# Autodesk Inventor assembly: painel
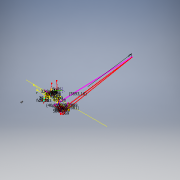
[picture p0: Inventor's stored thumbnail of the model, 180x180]
Saved by Autodesk Inventor 2019 (Build 230136000, 136)
## iProperties
Created: 2020-05-29
Part Number: painel
Document SubType Name: Assembly
Designer: luiza
_SolveAssemblyDoc: Frame Generator Solve Assembly
_Version: 15.0.0
Author: luiza
## Documents named in this file (8)
- G:\Meu Drive\Projetos\Projeto 2020 2021\Eletrônica 2020-2021\Projeção mecânica\Painel\old_painel.iam
- G:\Meu Drive\Projetos\Projeto 2020 2021\Eletrônica 2020-2021\Projeção mecânica\Painel\LCD12864_st7920.iam
- G:\Meu Drive\Projetos\Projeto 2020 2021\Eletrônica 2020-2021\Projeção mecânica\Painel\Tampa Painel.ipt
- G:\Meu Drive\Projetos\Projeto 2020 2021\Eletrônica 2020-2021\Projeção mecânica\Painel\Caixa Painel.ipt
- G:\Meu Drive\Projetos\Projeto 2020 2021\Eletrônica 2020-2021\Projeção mecânica\Painel\Espaçadores.ipt
- G:\Meu Drive\Projetos\Projeto 2020 2021\Suspensão & Direção 2020_2021\Geometrias\Geometria Suspensão e Direção.iam
- G:\Meu Drive\Projetos\Projeto 2020 2021\Eletrônica 2020-2021\Projeção mecânica\Painel\Fixação Painel.ipt
- G:\Meu Drive\Projetos\Projeto 2020 2021\Eletrônica 2020-2021\Projeção mecânica\Painel\painel\Frame\Frame0001.iam
## Components (11 placed, 7 different names)
1. LCD12864_st7920:1 [sub-assembly] — Flush:3, Mate:2, Mate:4, Mate:6
2. Tampa Painel:1 — Flush:3, Flush:4, Flush:5, Flush:7, Mate:1, Mate:3, Mate:5, Mate:7
3. Caixa Painel:1 — Flush:4, Flush:5, Mate:7, Mate:15, Mate:16
4. Espaçadores:1 — Flush:7
5. Espaçadores:2 — Mate:1, Mate:2
6. Espaçadores:3 — Mate:3, Mate:4
7. Espaçadores:4 — Mate:5, Mate:6
8. Geometria Suspensão e Direção:1 [sub-assembly] — Flush:8, Flush:9
9. Fixação Painel:1 — Flush:10, Flush:11, Mate:8, Mate:15, Mate:16
10. Fixação Painel:2 — Flush:10, Flush:11, Mate:8
11. Frame0001:1 [sub-assembly]
## Relationships (18: Mate 10, Flush 8)
- Flush:3: LCD12864_st7920:1 ↔ Tampa Painel:1
- Flush:4: Tampa Painel:1 ↔ Caixa Painel:1
- Flush:5: Tampa Painel:1 ↔ Caixa Painel:1
- Flush:7: Tampa Painel:1 ↔ Espaçadores:1
- Mate:1: Tampa Painel:1 ↔ Espaçadores:2
- Mate:2: LCD12864_st7920:1 ↔ Espaçadores:2
- Mate:3: Tampa Painel:1 ↔ Espaçadores:3
- Mate:4: LCD12864_st7920:1 ↔ Espaçadores:3
- Mate:5: Tampa Painel:1 ↔ Espaçadores:4
- Mate:6: LCD12864_st7920:1 ↔ Espaçadores:4
- Flush:8: Geometria Suspensão e Direção:1
- Flush:9: Geometria Suspensão e Direção:1
- Mate:7: Tampa Painel:1 ↔ Caixa Painel:1
- Flush:10: Fixação Painel:1 ↔ Fixação Painel:2
- Flush:11: Fixação Painel:1 ↔ Fixação Painel:2
- Mate:8 (150 mm): Fixação Painel:1 ↔ Fixação Painel:2
- Mate:15: Caixa Painel:1 ↔ Fixação Painel:1
- Mate:16: Caixa Painel:1 ↔ Fixação Painel:1
